# Autodesk Inventor assembly: MultiPass100V_outsideIn
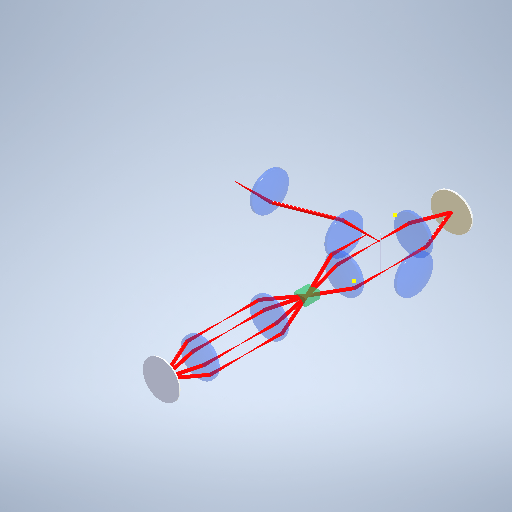
[picture p0: Inventor's stored thumbnail of the model, 512x512]
Saved by Autodesk Inventor 2026 (Build 300175050, 175E)
## iProperties
Created: 2024-08-19
Part Number: MultiPass100V_outsideIn
Document SubType Name: Assembly
Designer: User
Author: User
## Documents named in this file (15)
- C:\Users\newmanza\Documents\KerlinLab\Grants\EOD ROI 2025\MechanicalDrawingMultipass\MultiPass100V_outsideIn.iam
- C:\Users\newmanza\Documents\KerlinLab\Grants\EOD ROI 2025\MechanicalDrawingMultipass\BB1-E02-Solidworks.ipt
- C:\Users\newmanza\Documents\KerlinLab\Grants\EOD ROI 2025\MechanicalDrawingMultipass\LA1608-AB-Solidworks\LA1608-AB-Solidworks.ipt
- C:\Users\newmanza\Documents\KerlinLab\Grants\EOD ROI 2025\MechanicalDrawingMultipass\LaserBeamEntry1.ipt
- C:\Users\newmanza\Documents\KerlinLab\Grants\EOD ROI 2025\MechanicalDrawingMultipass\EntryMirror.ipt
- C:\Users\newmanza\Documents\KerlinLab\Grants\EOD ROI 2025\MechanicalDrawingMultipass\ExitMirror.ipt
- C:\Users\newmanza\Documents\KerlinLab\Grants\EOD ROI 2025\MechanicalDrawingMultipass\LaserBeamEntry2.ipt
- C:\Users\newmanza\Documents\KerlinLab\Grants\EOD ROI 2025\MechanicalDrawingMultipass\LaserBeamMirrorAngle1.ipt
- C:\Users\newmanza\Documents\KerlinLab\Grants\EOD ROI 2025\MechanicalDrawingMultipass\KTN1.ipt
- C:\Users\newmanza\Documents\KerlinLab\Grants\EOD ROI 2025\MechanicalDrawingMultipass\LaserBeamCenter3.ipt
- C:\Users\newmanza\Documents\KerlinLab\Grants\EOD ROI 2025\MechanicalDrawingMultipass\LaserBeamCenter4.ipt
- C:\Users\newmanza\Documents\KerlinLab\Grants\EOD ROI 2025\MechanicalDrawingMultipass\LaserBeam3x.ipt
- C:\Users\newmanza\Documents\KerlinLab\Grants\EOD ROI 2025\MechanicalDrawingMultipass\LoopPlane1.ipt
- C:\Users\newmanza\Documents\KerlinLab\Grants\EOD ROI 2025\MechanicalDrawingMultipass\LaserBeamMirrorAngle2.ipt
- C:\Users\newmanza\Documents\KerlinLab\Grants\EOD ROI 2025\MechanicalDrawingMultipass\LaserBeamEntry2x.ipt
## Components (50 placed, 14 different names)
1. BB1-E02-Solidworks:1 — Mate:15, Mate:16, Mate:17, Mate:150, Mate:154, Mate:224
2. BB1-E02-Solidworks:2 — Mate:13, Mate:14, Mate:18, Mate:126, Mate:136, Mate:182, Mate:186, Mate:244, Mate:248
3. LA1608-AB-Solidworks:1 — Mate:5, Mate:6, Mate:7, Mate:8, Mate:11, Mate:12, Mate:106, Mate:110, Mate:111, Mate:120, Mate:122, Mate:130, Mate:132, Mate:171, Mate:174, Mate:175, Mate:177, Mate:190, Mate:194, Mate:195, Mate:235, Mate:236, Mate:237
4. LA1608-AB-Solidworks:3 — Mate:27, Mate:28, Mate:209, Mate:210, Mate:211, Flush:242, Mate:241, Mate:242
5. LA1608-AB-Solidworks:4 — Mate:7, Mate:8, Mate:12, Mate:13, Mate:14, Mate:18, Mate:119, Mate:124, Mate:125, Mate:129, Mate:134, Mate:135, Mate:172, Mate:173, Mate:176, Mate:181, Mate:185, Mate:189, Mate:223, Mate:238, Mate:245, Mate:249
6. LA1608-AB-Solidworks:5 — Mate:3, Mate:4, Mate:5, Mate:6, Mate:10, Mate:11, Mate:21, Mate:43, Flush:7, Mate:104, Mate:105, Mate:107, Mate:113, Mate:143, Mate:158, Mate:162, Mate:163, Mate:199, Mate:203, Mate:204, Mate:230, Mate:231, Mate:232, Mate:233, Mate:234
7. LA1608-AB-Solidworks:6 — Mate:3, Mate:4, Mate:10, Mate:15, Mate:16, Mate:17, Mate:19, Mate:20, Flush:1, Flush:5, Mate:38, Mate:41, Mate:42, Mate:144, Mate:147, Mate:149, Mate:152, Mate:153, Mate:157, Mate:161, Mate:225, Mate:239
8. LA1608-AB-Solidworks:7 — Mate:29, Flush:2, Mate:30, Mate:31, Flush:3
9. LaserBeamEntry1:1 — Mate:30, Mate:31
10. LaserBeamEntry1:2 — Mate:38, Flush:6
11. EntryMirror:1
12. LaserBeamEntry2:1 — Mate:35, Flush:3
13. LaserBeamEntry2:2 — Mate:37, Flush:5, Flush:6
14. LaserBeamEntry2:3 — Mate:41, Mate:42
15. LaserBeamEntry2:4 — Mate:43, Flush:7
16. LaserBeamEntry2:5 — Mate:131, Mate:132
17. LaserBeamEntry2:6 — Mate:145, Mate:233
18. LaserBeamEntry2:8 — Mate:123, Mate:124, Mate:128
19. LaserBeamEntry2:9 — Mate:121, Mate:122
20. LaserBeamEntry2:10 — Mate:173, Mate:176, Mate:251
21. LaserBeamEntry2:11 — Mate:146, Mate:147
22. LaserBeamMirrorAngle1:1 — Mate:127, Mate:128
23. LaserBeamMirrorAngle1:2 — Mate:137, Mate:238
24. LaserBeamMirrorAngle1:3 — Mate:151, Mate:152
25. LaserBeamMirrorAngle1:4 — Mate:155, Mate:239
26. LaserBeamEntry2:12 — Mate:174, Mate:175
27. LaserBeamEntry2:13 — Mate:133, Mate:134
28. LaserBeamEntry2:14 — Mate:160, Mate:162
29. LaserBeamEntry2:15 — Mate:159, Mate:161
30. LaserBeamEntry2:17 — Mate:191, Mate:223, Mate:247
31. LaserBeamEntry2:18 — Mate:193, Mate:194
32. ExitMirror:2
33. KTN1:1 — Mate:104, Mate:105, Mate:106, Mate:108, Mate:109, Mate:112, Mate:114, Mate:118, Mate:164, Mate:178, Mate:196, Mate:200, Mate:220
34. LaserBeamCenter3:1 — Mate:115, Mate:231
35. LaserBeamCenter3:2 — Mate:117, Mate:118
36. LaserBeamCenter3:3 — Mate:139, Mate:237
37. LaserBeamCenter3:4 — Mate:141, Mate:232
38. LaserBeamCenter3:5 — Mate:165, Mate:230
39. LaserBeamCenter4:1 — Mate:179, Mate:235
40. LaserBeamCenter4:4 — Mate:197, Mate:236
41. LaserBeamCenter4:5 — Mate:201, Mate:234
42. LaserBeamEntry2:20 — Mate:203, Mate:204, Mate:243
43. LA1608-AB-Solidworks:8 — Mate:209, Mate:210, Mate:212, Mate:216, Mate:217, Flush:242
44. LaserBeamEntry2:21 — Mate:216, Mate:217
45. LaserBeam3x:1 — Mate:218, Mate:241
46. LoopPlane1:1 — Mate:220, Mate:221
47. LaserBeamMirrorAngle1:5 — Mate:224, Mate:225
48. LaserBeamMirrorAngle2:1 — Mate:250, Mate:251
49. LaserBeamMirrorAngle2:2 — Mate:246, Mate:247
50. LaserBeamEntry2x:1 — Mate:242, Mate:243
## Relationships (155: Mate 148, Flush 7)
- Mate:3: LA1608-AB-Solidworks:5 ↔ LA1608-AB-Solidworks:6
- Mate:4 (-50 mm): LA1608-AB-Solidworks:5 ↔ LA1608-AB-Solidworks:6
- Mate:5: LA1608-AB-Solidworks:1 ↔ LA1608-AB-Solidworks:5
- Mate:6 (50 mm): LA1608-AB-Solidworks:1 ↔ LA1608-AB-Solidworks:5
- Mate:7: LA1608-AB-Solidworks:1 ↔ LA1608-AB-Solidworks:4
- Mate:8 (-50 mm): LA1608-AB-Solidworks:1 ↔ LA1608-AB-Solidworks:4
- Mate:10: LA1608-AB-Solidworks:5 ↔ LA1608-AB-Solidworks:6
- Mate:11: LA1608-AB-Solidworks:1 ↔ LA1608-AB-Solidworks:5
- Mate:12: LA1608-AB-Solidworks:1 ↔ LA1608-AB-Solidworks:4
- Mate:13: BB1-E02-Solidworks:2 ↔ LA1608-AB-Solidworks:4
- Mate:14 (25 mm): BB1-E02-Solidworks:2 ↔ LA1608-AB-Solidworks:4
- Mate:15: BB1-E02-Solidworks:1 ↔ LA1608-AB-Solidworks:6
- Mate:16 (-25 mm): BB1-E02-Solidworks:1 ↔ LA1608-AB-Solidworks:6
- Mate:17: BB1-E02-Solidworks:1 ↔ LA1608-AB-Solidworks:6
- Mate:18: BB1-E02-Solidworks:2 ↔ LA1608-AB-Solidworks:4
- Mate:19: LA1608-AB-Solidworks:6
- Mate:20: LA1608-AB-Solidworks:6
- Mate:21: LA1608-AB-Solidworks:5
- Mate:22
- Mate:23
- Flush:1 (-25 mm): LA1608-AB-Solidworks:6
- Mate:24
- Mate:25
- Mate:27: LA1608-AB-Solidworks:3
- Mate:28 (-34 mm): LA1608-AB-Solidworks:3
- Mate:29: LA1608-AB-Solidworks:7
- Flush:2 (-25 mm): LA1608-AB-Solidworks:7
- Mate:30: LA1608-AB-Solidworks:7 ↔ LaserBeamEntry1:1
- Mate:31: LA1608-AB-Solidworks:7 ↔ LaserBeamEntry1:1
- Mate:35: LaserBeamEntry2:1
- Flush:3: LA1608-AB-Solidworks:7 ↔ LaserBeamEntry2:1
- Mate:37: LaserBeamEntry2:2
- Flush:5: LA1608-AB-Solidworks:6 ↔ LaserBeamEntry2:2
- Mate:38: LA1608-AB-Solidworks:6 ↔ LaserBeamEntry1:2
- Flush:6: LaserBeamEntry1:2 ↔ LaserBeamEntry2:2
- Mate:41: LA1608-AB-Solidworks:6 ↔ LaserBeamEntry2:3
- Mate:42: LA1608-AB-Solidworks:6 ↔ LaserBeamEntry2:3
- Mate:43: LA1608-AB-Solidworks:5 ↔ LaserBeamEntry2:4
- Flush:7: LA1608-AB-Solidworks:5 ↔ LaserBeamEntry2:4
- Mate:104: LA1608-AB-Solidworks:5 ↔ KTN1:1
- Mate:105 (25 mm): LA1608-AB-Solidworks:5 ↔ KTN1:1
- Mate:106: LA1608-AB-Solidworks:1 ↔ KTN1:1
- Mate:107: LA1608-AB-Solidworks:5
- Mate:108: KTN1:1
- Mate:109: KTN1:1
- Mate:110: LA1608-AB-Solidworks:1
- Mate:111: LA1608-AB-Solidworks:1
- Mate:112: KTN1:1
- Mate:113: LA1608-AB-Solidworks:5
- Mate:114: KTN1:1
- Mate:115: LaserBeamCenter3:1
- Mate:117: LaserBeamCenter3:2
- Mate:118: KTN1:1 ↔ LaserBeamCenter3:2
- Mate:119: LA1608-AB-Solidworks:4
- Mate:120: LA1608-AB-Solidworks:1
- Mate:121: LaserBeamEntry2:9
- Mate:122: LA1608-AB-Solidworks:1 ↔ LaserBeamEntry2:9
- Mate:123: LaserBeamEntry2:8
- Mate:124: LA1608-AB-Solidworks:4 ↔ LaserBeamEntry2:8
- Mate:125: LA1608-AB-Solidworks:4
- Mate:126: BB1-E02-Solidworks:2
- Mate:127: LaserBeamMirrorAngle1:1
- Mate:128 (0.2 mm): LaserBeamEntry2:8 ↔ LaserBeamMirrorAngle1:1
- Mate:129: LA1608-AB-Solidworks:4
- Mate:130: LA1608-AB-Solidworks:1
- Mate:131: LaserBeamEntry2:5
- Mate:132: LA1608-AB-Solidworks:1 ↔ LaserBeamEntry2:5
- Mate:133: LaserBeamEntry2:13
- Mate:134: LA1608-AB-Solidworks:4 ↔ LaserBeamEntry2:13
- Mate:135: LA1608-AB-Solidworks:4
- Mate:136: BB1-E02-Solidworks:2
- Mate:137: LaserBeamMirrorAngle1:2
- Mate:139: LaserBeamCenter3:3
- Mate:141: LaserBeamCenter3:4
- Mate:143: LA1608-AB-Solidworks:5
- Mate:144: LA1608-AB-Solidworks:6
- Mate:145: LaserBeamEntry2:6
- Mate:146: LaserBeamEntry2:11
- Mate:147: LA1608-AB-Solidworks:6 ↔ LaserBeamEntry2:11
- Mate:149: LA1608-AB-Solidworks:6
- Mate:150: BB1-E02-Solidworks:1
- Mate:151: LaserBeamMirrorAngle1:3
- Mate:152 (0.2 mm): LA1608-AB-Solidworks:6 ↔ LaserBeamMirrorAngle1:3
- Mate:153: LA1608-AB-Solidworks:6
- Mate:154: BB1-E02-Solidworks:1
- Mate:155: LaserBeamMirrorAngle1:4
- Mate:157: LA1608-AB-Solidworks:6
- Mate:158: LA1608-AB-Solidworks:5
- Mate:159: LaserBeamEntry2:15
- Mate:160: LaserBeamEntry2:14
- Mate:161: LA1608-AB-Solidworks:6 ↔ LaserBeamEntry2:15
- Mate:162: LA1608-AB-Solidworks:5 ↔ LaserBeamEntry2:14
- Mate:163: LA1608-AB-Solidworks:5
- Mate:164: KTN1:1
- Mate:165: LaserBeamCenter3:5
- Mate:171: LA1608-AB-Solidworks:1
- Mate:172: LA1608-AB-Solidworks:4
- Mate:173: LA1608-AB-Solidworks:4 ↔ LaserBeamEntry2:10
- Mate:174: LA1608-AB-Solidworks:1 ↔ LaserBeamEntry2:12
- Mate:175: LA1608-AB-Solidworks:1 ↔ LaserBeamEntry2:12
- Mate:176: LA1608-AB-Solidworks:4 ↔ LaserBeamEntry2:10
- Mate:177: LA1608-AB-Solidworks:1
- Mate:178: KTN1:1
- Mate:179: LaserBeamCenter4:1
- Mate:181: LA1608-AB-Solidworks:4
- Mate:182: BB1-E02-Solidworks:2
- Mate:185: LA1608-AB-Solidworks:4
- Mate:186: BB1-E02-Solidworks:2
- Mate:189: LA1608-AB-Solidworks:4
- Mate:190: LA1608-AB-Solidworks:1
- Mate:191: LaserBeamEntry2:17
- Mate:193: LaserBeamEntry2:18
- Mate:194: LA1608-AB-Solidworks:1 ↔ LaserBeamEntry2:18
- Mate:195: LA1608-AB-Solidworks:1
- Mate:196: KTN1:1
- Mate:197: LaserBeamCenter4:4
- Mate:199: LA1608-AB-Solidworks:5
- Mate:200: KTN1:1
- Mate:201: LaserBeamCenter4:5
- Mate:203: LA1608-AB-Solidworks:5 ↔ LaserBeamEntry2:20
- Mate:204: LA1608-AB-Solidworks:5 ↔ LaserBeamEntry2:20
- Mate:209: LA1608-AB-Solidworks:3 ↔ LA1608-AB-Solidworks:8
- Mate:210 (50 mm): LA1608-AB-Solidworks:3 ↔ LA1608-AB-Solidworks:8
- Mate:211: LA1608-AB-Solidworks:3
- Mate:212: LA1608-AB-Solidworks:8
- Mate:216: LA1608-AB-Solidworks:8 ↔ LaserBeamEntry2:21
- Mate:217: LA1608-AB-Solidworks:8 ↔ LaserBeamEntry2:21
- Mate:218: LaserBeam3x:1
- Mate:220: KTN1:1 ↔ LoopPlane1:1
- Mate:221: LoopPlane1:1
- Mate:223: LA1608-AB-Solidworks:4 ↔ LaserBeamEntry2:17
- Mate:224: BB1-E02-Solidworks:1 ↔ LaserBeamMirrorAngle1:5
- Mate:225 (-0.2 mm): LA1608-AB-Solidworks:6 ↔ LaserBeamMirrorAngle1:5
- Mate:230 (-0.2 mm): LA1608-AB-Solidworks:5 ↔ LaserBeamCenter3:5
- Mate:231 (-0.2 mm): LA1608-AB-Solidworks:5 ↔ LaserBeamCenter3:1
- Mate:232 (-0.2 mm): LA1608-AB-Solidworks:5 ↔ LaserBeamCenter3:4
- Mate:233: LA1608-AB-Solidworks:5 ↔ LaserBeamEntry2:6
- Mate:234 (-0.3 mm): LA1608-AB-Solidworks:5 ↔ LaserBeamCenter4:5
- Mate:235 (-0.3 mm): LA1608-AB-Solidworks:1 ↔ LaserBeamCenter4:1
- Mate:236 (-0.3 mm): LA1608-AB-Solidworks:1 ↔ LaserBeamCenter4:4
- Mate:237 (-0.3 mm): LA1608-AB-Solidworks:1 ↔ LaserBeamCenter3:3
- Mate:238 (-0.2 mm): LA1608-AB-Solidworks:4 ↔ LaserBeamMirrorAngle1:2
- Mate:239 (-0.2 mm): LA1608-AB-Solidworks:6 ↔ LaserBeamMirrorAngle1:4
- Flush:242: LA1608-AB-Solidworks:3 ↔ LA1608-AB-Solidworks:8
- Mate:241 (-0.1 mm): LA1608-AB-Solidworks:3 ↔ LaserBeam3x:1
- Mate:242: LA1608-AB-Solidworks:3 ↔ LaserBeamEntry2x:1
- Mate:243: LaserBeamEntry2:20 ↔ LaserBeamEntry2x:1
- Mate:244: BB1-E02-Solidworks:2
- Mate:245: LA1608-AB-Solidworks:4
- Mate:246: LaserBeamMirrorAngle2:2
- Mate:247 (0.1 mm): LaserBeamEntry2:17 ↔ LaserBeamMirrorAngle2:2
- Mate:248: BB1-E02-Solidworks:2
- Mate:249: LA1608-AB-Solidworks:4
- Mate:250: LaserBeamMirrorAngle2:1
- Mate:251 (0.15 mm): LaserBeamEntry2:10 ↔ LaserBeamMirrorAngle2:1
